# Autodesk Inventor assembly: 000 ASY GBK Gubkinskiy
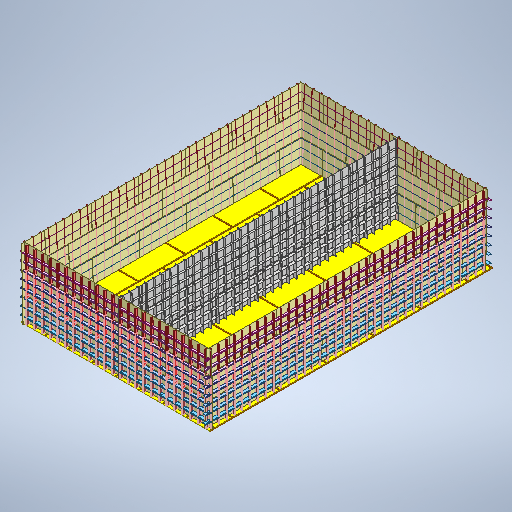
[picture p0: Inventor's stored thumbnail of the model, 512x512]
Saved by Autodesk Inventor 2026.2 (Build 302298000, 298)
## iProperties
Created: 2026-04-17
Part Number: 000 ASY GBK Gubkinskiy
Document SubType Name: Assembly
Designer: admin
Author: admin
## Documents named in this file (11)
- C:\Users\admin\Documents\Inventor\GBK-Gubkinskiy\000 ASY GBK Gubkinskiy.iam
- C:\Users\admin\Documents\Inventor\GBK-Gubkinskiy\GBK bottom.ipt
- C:\Users\admin\Documents\Inventor\GBK-Gubkinskiy\GBK dummy wall 1.ipt
- C:\Users\admin\Documents\Inventor\GBK-Gubkinskiy\GBK dummy wall 4.ipt
- C:\Users\admin\Documents\Inventor\GBK-Gubkinskiy\GBK overall model.ipt
- C:\Users\admin\Documents\Inventor\GBK-Gubkinskiy\0401 ASY GBK wall shield Center 1.iam
- C:\Users\admin\Documents\Inventor\GBK-Gubkinskiy\0701 ASY GBK wall shield Center 4.iam
- C:\Users\admin\Documents\Inventor\GBK-Gubkinskiy\01001 ASY GBK wall shield Center 10.iam
- C:\Users\admin\Documents\Inventor\GBK-Gubkinskiy\ASY GBK правая стенка.iam
- C:\Users\admin\Documents\Inventor\GBK-Gubkinskiy\ASY GBK предварительная торцевая.iam
- C:\Users\admin\Documents\Inventor\GBK-Gubkinskiy\090 ASY bottom.iam
## Components (46 placed, 10 different names)
1. GBK bottom.ipt:1 — Mate:10, Mate:11, Mate:12, Mate:13, Mate:14, Rigid:1, Flush:4, Flush:6, Flush:7, Flush:8
2. GBK dummy wall 1.ipt:1 — Mate:10
3. GBK dummy wall 1.ipt:2 — Mate:11, Mate:12
4. GBK dummy wall 4.ipt:1 — Mate:13, Mate:14
5. GBK overall model:1 — Rigid:1
6. ASY GBK правая стенка:1 [sub-assembly]
7. ASY GBK предварительная торцевая:1 [sub-assembly]
8. ASY GBK предварительная торцевая:2 [sub-assembly] — Mate:17, Flush:4
9. ASY GBK правая стенка:2 [sub-assembly] — Flush:5, Flush:6
10. 090 ASY bottom:1 [sub-assembly] — Mate:19, Flush:8
11. 0401 ASY GBK wall shield Center 1:1 [sub-assembly] — Rigid:2, Mate:18, Flush:7
12. 01001 ASY GBK wall shield Center 10:1 [sub-assembly] — Rigid:3
13. 0701 ASY GBK wall shield Center 4:1 [sub-assembly] — Rigid:2, Rigid:3
14. 0401 ASY GBK wall shield Center 1:2 [sub-assembly]
15. 01001 ASY GBK wall shield Center 10:2 [sub-assembly]
16. 0701 ASY GBK wall shield Center 4:2 [sub-assembly]
17. 0401 ASY GBK wall shield Center 1:3 [sub-assembly]
18. 01001 ASY GBK wall shield Center 10:3 [sub-assembly]
19. 0701 ASY GBK wall shield Center 4:3 [sub-assembly]
20. 0401 ASY GBK wall shield Center 1:4 [sub-assembly]
21. 01001 ASY GBK wall shield Center 10:4 [sub-assembly]
22. 0701 ASY GBK wall shield Center 4:4 [sub-assembly]
23. 0401 ASY GBK wall shield Center 1:5 [sub-assembly]
24. 01001 ASY GBK wall shield Center 10:5 [sub-assembly]
25. 0701 ASY GBK wall shield Center 4:5 [sub-assembly]
26. 0401 ASY GBK wall shield Center 1:6 [sub-assembly]
27. 01001 ASY GBK wall shield Center 10:6 [sub-assembly]
28. 0701 ASY GBK wall shield Center 4:6 [sub-assembly]
29. 0401 ASY GBK wall shield Center 1:7 [sub-assembly]
30. 01001 ASY GBK wall shield Center 10:7 [sub-assembly]
31. 0701 ASY GBK wall shield Center 4:7 [sub-assembly]
32. 0401 ASY GBK wall shield Center 1:8 [sub-assembly]
33. 01001 ASY GBK wall shield Center 10:8 [sub-assembly]
34. 0701 ASY GBK wall shield Center 4:8 [sub-assembly]
35. 0401 ASY GBK wall shield Center 1:9 [sub-assembly]
36. 01001 ASY GBK wall shield Center 10:9 [sub-assembly]
37. 0701 ASY GBK wall shield Center 4:9 [sub-assembly]
38. 0401 ASY GBK wall shield Center 1:10 [sub-assembly]
39. 01001 ASY GBK wall shield Center 10:10 [sub-assembly]
40. 0701 ASY GBK wall shield Center 4:10 [sub-assembly]
41. 0401 ASY GBK wall shield Center 1:11 [sub-assembly]
42. 01001 ASY GBK wall shield Center 10:11 [sub-assembly]
43. 0701 ASY GBK wall shield Center 4:11 [sub-assembly]
44. 0401 ASY GBK wall shield Center 1:12 [sub-assembly]
45. 01001 ASY GBK wall shield Center 10:12 [sub-assembly]
46. 0701 ASY GBK wall shield Center 4:12 [sub-assembly]
## Component patterns: (12 elements, first: 0401 ASY GBK wall shield Center 1:1 + 01001 ASY GBK wall shield Center 10:1 + 0701 ASY GBK wall shield Center 4:1)
## Relationships (20: Mate 10, Flush 7, WeldJoint 3)
- [Flush]: GBK bottom.ipt:1 ↔ ASY GBK правая стенка:1
- [Mate]: GBK bottom.ipt:1 ↔ ASY GBK правая стенка:1
- Mate:10: GBK bottom.ipt:1 ↔ GBK dummy wall 1.ipt:1
- Mate:11: GBK bottom.ipt:1 ↔ GBK dummy wall 1.ipt:2
- Mate:12: GBK bottom.ipt:1 ↔ GBK dummy wall 1.ipt:2
- Mate:13: GBK bottom.ipt:1 ↔ GBK dummy wall 4.ipt:1
- Mate:14: GBK bottom.ipt:1 ↔ GBK dummy wall 4.ipt:1
- Rigid:1 [WeldJoint]: GBK bottom.ipt:1 ↔ GBK overall model:1
- [Mate]: ASY GBK предварительная торцевая:1
- [Flush]: GBK bottom.ipt:1 ↔ ASY GBK предварительная торцевая:1
- Mate:17: ASY GBK предварительная торцевая:2
- Flush:4: GBK bottom.ipt:1 ↔ ASY GBK предварительная торцевая:2
- Flush:5: ASY GBK правая стенка:2
- Flush:6: GBK bottom.ipt:1 ↔ ASY GBK правая стенка:2
- Rigid:2 [WeldJoint]: 0401 ASY GBK wall shield Center 1:1 ↔ 0701 ASY GBK wall shield Center 4:1
- Rigid:3 [WeldJoint]: 01001 ASY GBK wall shield Center 10:1 ↔ 0701 ASY GBK wall shield Center 4:1
- Mate:18: 0401 ASY GBK wall shield Center 1:1
- Flush:7: GBK bottom.ipt:1 ↔ 0401 ASY GBK wall shield Center 1:1
- Mate:19: 090 ASY bottom:1
- Flush:8: GBK bottom.ipt:1 ↔ 090 ASY bottom:1
## Named parameters: Зазор_по_горизонту = 1 mm, d120_Зазор_по_горизонту = 1 mm, d141_Зазор_по_горизонту = 1 mm, d159_d141_Зазор_по_горизонту = 1 mm, d175_d141_Зазор_по_горизонту = 1 mm
